# Autodesk Inventor assembly: HS 24T Gear, Circle_mirrored
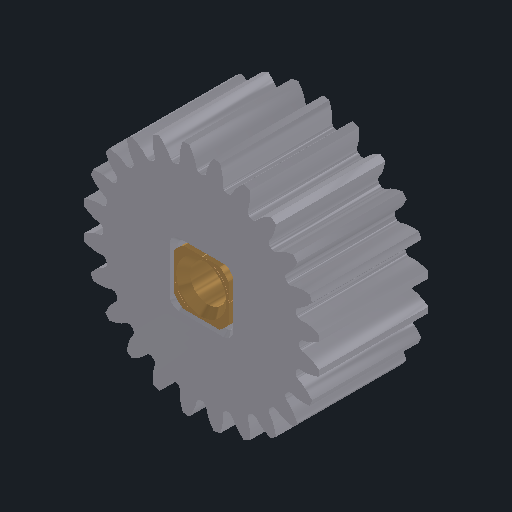
[picture p0: Inventor's stored thumbnail of the model, 512x512]
Saved by Autodesk Inventor 2025 (Build 290162000, 162)
## iProperties
Created: 2022-08-02
Part Number: HS 24T Gear, Circle_mirrored
Document SubType Name: Assembly
Designer: Averey Ku
Author: ylu12
## Documents named in this file (3)
- D:\vex_robotics_high_stakes\hardware\cad\bots\high_stakes_v2\chassis_v2\drivebay_mirrored\HS 24T Gear, Circle_mirrored.iam
- D:\vex_robotics_high_stakes\hardware\cad\bots\high_stakes_v2\chassis_v2\drivebay_mirrored\HS Shaft Adapter Circle_mirrored.ipt
- D:\vex_robotics_high_stakes\hardware\cad\bots\high_stakes_v2\chassis_v2\drivebay_mirrored\HS 24T Gear, No Insert_mirrored.ipt
## Components (2 placed, 2 different names)
1. HS Shaft Adapter Circle_mirrored:1 — Flush:1, Mate:2, Mate:1
2. HS 24T Gear, No Insert_mirrored:1 — Flush:4, Mate:8, Mate:7
## Relationships (6: Mate 4, Flush 2)
- Flush:1 (-6.35 mm): HS Shaft Adapter Circle_mirrored:1
- Mate:2: HS Shaft Adapter Circle_mirrored:1
- Mate:1: HS Shaft Adapter Circle_mirrored:1
- Flush:4: HS 24T Gear, No Insert_mirrored:1
- Mate:8: HS 24T Gear, No Insert_mirrored:1
- Mate:7: HS 24T Gear, No Insert_mirrored:1
